# Autodesk Inventor assembly: IMX178 Camera Case Assembly
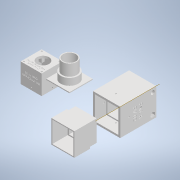
[picture p0: Inventor's stored thumbnail of the model, 180x180]
Saved by Autodesk Inventor 2022.1 (Build 261234000, 234)
## iProperties
Created: 2021-07-25
Part Number: IMX178 Camera Case Assembly
Document SubType Name: Assembly
Designer: robst
Author: robst
## Documents named in this file (6)
- C:\git\CAD-Development\robSteele\ShapeWays\GlobalMeteorNetwork\IMX178 Camera Case Assembly.iam
- C:\git\CAD-Development\robSteele\ShapeWays\GlobalMeteorNetwork\IMX178 Camera Case Telescope Attachement.ipt
- C:\git\CAD-Development\robSteele\ShapeWays\GlobalMeteorNetwork\IMX178 Camera Case Bottom.ipt
- C:\git\CAD-Development\robSteele\ShapeWays\GlobalMeteorNetwork\IMX178 Camera Case.ipt
- C:\git\CAD-Development\robSteele\ShapeWays\GlobalMeteorNetwork\IMX178 Camera Case Cap.ipt
- C:\git\CAD-Development\robSteele\ShapeWays\GlobalMeteorNetwork\IMX178 Shell For Ethernet Strain Relief.ipt
## Components (5 placed, 5 different names)
1. IMX178 Camera Case:1 — Mate:1, Flush:1, Flush:2
2. IMX178 Camera Case Telescope Attachement:1
3. IMX178 Camera Case Bottom:1 — Mate:1, Flush:1, Flush:2
4. IMX178 Camera Case Cap:1
5. IMX178 Shell For Ethernet Strain Relief:1
## Relationships (3: Flush 2, Mate 1)
- Mate:1: IMX178 Camera Case:1 ↔ IMX178 Camera Case Bottom:1
- Flush:1: IMX178 Camera Case:1 ↔ IMX178 Camera Case Bottom:1
- Flush:2: IMX178 Camera Case:1 ↔ IMX178 Camera Case Bottom:1
